# Autodesk Inventor assembly: 100-10-FRAME-PROFILE-BOT-H-01
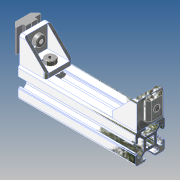
[picture p0: Inventor's stored thumbnail of the model, 180x180]
Saved by Autodesk Inventor 2018.2 (Build 222227000, 227)
## iProperties
Manager: feesmrt
Company: FRANCOR
Part Number: 100-10-FRAME-PROFILE-BOT-H-01
Project: Rescue Robot
Cost Center: -
Material: Generisch
Document SubType Name: Assembly
Designer: feesmrt
Engineer: feesmrt
Authority: feesmrt
Subject: Rescue Robot
Author: feesmrt
Revision Number: 1
## Documents named in this file (4)
- D:\Programmierung\FRANC0R\CAD\02-Rocker-Bogie-Robot\100-CHASSIS\10-FRAME\100-10-FRAME-PROFILE-BOT-H-01.iam
- D:\Programmierung\FRANC0R\CAD\02-Rocker-Bogie-Robot\100-CHASSIS\10-FRAME\100-10-FRAME-PROFILE-BOT-H-01.ipt
- D:\Programmierung\FRANC0R\CAD\02-Rocker-Bogie-Robot\900-COMPONENTS\900-50-PROFILES\900-50-PROFILES-ANGLE-CONN-20x20-01.iam
- D:\Programmierung\FRANC0R\CAD\02-Rocker-Bogie-Robot\900-COMPONENTS\900-50-PROFILES\900-50-PROFILES-ANGLE-CONN-20x20-01-N6_N8.iam
## Components (3 placed, 3 different names)
1. 100-10-FRAME-PROFILE-BOT-H-01:1 — Passend:2, Fluchtend:4, Passend:4, Fluchtend:5, Passend:5
2. 900-50-PROFILES-ANGLE-CONN-20x20-01:2 [sub-assembly] — Passend:2, Fluchtend:4, Passend:3
3. 900-50-PROFILES-ANGLE-CONN-20x20-01-N6_N8:1 [sub-assembly] — Passend:4, Fluchtend:5, Passend:5
## Relationships (6: Mate 4, Flush 2)
- Passend:2 [Mate]: 100-10-FRAME-PROFILE-BOT-H-01:1 ↔ 900-50-PROFILES-ANGLE-CONN-20x20-01:2
- Fluchtend:4 [Flush]: 100-10-FRAME-PROFILE-BOT-H-01:1 ↔ 900-50-PROFILES-ANGLE-CONN-20x20-01:2
- Passend:3 [Mate]: 900-50-PROFILES-ANGLE-CONN-20x20-01:2
- Passend:4 [Mate]: 100-10-FRAME-PROFILE-BOT-H-01:1 ↔ 900-50-PROFILES-ANGLE-CONN-20x20-01-N6_N8:1
- Fluchtend:5 [Flush]: 100-10-FRAME-PROFILE-BOT-H-01:1 ↔ 900-50-PROFILES-ANGLE-CONN-20x20-01-N6_N8:1
- Passend:5 [Mate]: 100-10-FRAME-PROFILE-BOT-H-01:1 ↔ 900-50-PROFILES-ANGLE-CONN-20x20-01-N6_N8:1
